# Autodesk Inventor assembly: copy2
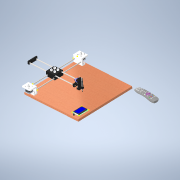
[picture p0: Inventor's stored thumbnail of the model, 180x180]
Saved by Autodesk Inventor 2021 (Build 250183000, 183)
## iProperties
Created: 2021-07-13
Part Number: copy2
Document SubType Name: Assembly
Designer: Michael Swaminathan
Author: Michael Swaminathan
## Documents named in this file (20)
- F:\Pattern Drawing Bot\Xy plotter Drawing Machine\XY Plotter Drawing Machine.iam
- F:\Pattern Drawing Bot\Xy plotter Drawing Machine\base.ipt
- F:\Pattern Drawing Bot\Xy plotter Drawing Machine\Display Controller LCD.ipt
- F:\Pattern Drawing Bot\Xy plotter Drawing Machine\Buzzer.ipt
- F:\Pattern Drawing Bot\Xy plotter Drawing Machine\Motor With Support Assembly.iam
- F:\Pattern Drawing Bot\Xy plotter Drawing Machine\Guidance Rods 2.ipt
- F:\Pattern Drawing Bot\Xy plotter Drawing Machine\Central Portion Assembly.iam
- F:\Pattern Drawing Bot\Xy plotter Drawing Machine\Y-Axis.ipt
- F:\Pattern Drawing Bot\Xy plotter Drawing Machine\Y-axis on Holder.ipt
- F:\Pattern Drawing Bot\Xy plotter Drawing Machine\Screw(2).ipt
- F:\Pattern Drawing Bot\Xy plotter Drawing Machine\Guidance Rods.ipt
- F:\Pattern Drawing Bot\Xy plotter Drawing Machine\Pen Holder.ipt
- F:\Pattern Drawing Bot\Xy plotter Drawing Machine\Holding Stand.ipt
- F:\Pattern Drawing Bot\Xy plotter Drawing Machine\BIC Round Stic Pen Assembly.iam
- F:\Pattern Drawing Bot\Xy plotter Drawing Machine\Servo Motor Support.ipt
- F:\Pattern Drawing Bot\Xy plotter Drawing Machine\Servo motor support rods.ipt
- F:\Pattern Drawing Bot\Xy plotter Drawing Machine\Micro Servo SG90.ipt
- F:\Pattern Drawing Bot\Xy plotter Drawing Machine\Rollers(2).ipt
- F:\Pattern Drawing Bot\Xy plotter Drawing Machine\roller support on y axis.ipt
- F:\Pattern Drawing Bot\Xy plotter Drawing Machine\remote controller.ipt
## Components (28 placed, 19 different names)
1. base:1 — Rigid:1, Rotational:1, Rotational:2, Rotational:3
2. Display Controller LCD:1 — Rigid:1, Rotational:4, Rotational:6, Rotational:7, Rotational:11
3. Buzzer:1 — Rotational:1
4. Motor With Support Assembly:1 [sub-assembly] — Rotational:2, Rigid:2, Rigid:3
5. Motor With Support Assembly:2 [sub-assembly] — Rotational:3, Mate:3, Mate:4
6. Guidance Rods 2:1 — Rigid:3, Mate:1, Mate:4
7. Guidance Rods 2:2 — Rigid:2, Insert:1, Mate:3
8. Central Portion Assembly:1 [sub-assembly] — Insert:1, Mate:1, Insert:2, Mate:5
9. Guidance Rods 2:3 — Mate:5, Insert:6, Mate:8
10. Guidance Rods 2:4 — Insert:2, Insert:5, Insert:12
11. Y-Axis:1 — Insert:12, Mate:8
12. Y-axis on Holder:1 — Insert:5, Insert:6, Rigid:4, Rigid:5, Rigid:12, Insert:8, Mate:7, Insert:10
13. Screw(2):1 — Rotational:11
14. Screw(2):2 — Rotational:4
15. Screw(2):3 — Rotational:6
16. Screw(2):4 — Rotational:7
17. Guidance Rods:1 — Rigid:4, Insert:7
18. Guidance Rods:2 — Rigid:5, Mate:6
19. Pen Holder:1 — Rigid:13, Insert:9
20. Holding Stand:1 — Mate:6, Insert:7, Insert:9
21. BIC Round Stic Pen Assembly:1 [sub-assembly] — Rigid:13
22. Servo Motor Support:1 — Rotational:10
23. Servo motor support rods:1 — Rigid:12, Rotational:10
24. Servo motor support rods:2 — Insert:8
25. Micro Servo SG90:1 — Mate:7
26. Rollers(2):1 — Insert:11
27. roller support on y axis:1 — Insert:10, Insert:11
28. remote controller:1
## Relationships (32: Insert 10, RevoluteJoint 8, WeldJoint 7, Mate 7)
- Rigid:1 [WeldJoint]: base:1 ↔ Display Controller LCD:1
- Rotational:1 [RevoluteJoint]: base:1 ↔ Buzzer:1
- Rotational:2 [RevoluteJoint]: base:1 ↔ Motor With Support Assembly:1
- Rotational:3 [RevoluteJoint]: base:1 ↔ Motor With Support Assembly:2
- Rigid:2 [WeldJoint] (-6 mm): Motor With Support Assembly:1 ↔ Guidance Rods 2:2
- Rigid:3 [WeldJoint] (-4 mm): Motor With Support Assembly:1 ↔ Guidance Rods 2:1
- Insert:1 (-250 mm): Guidance Rods 2:2 ↔ Central Portion Assembly:1
- Mate:1: Guidance Rods 2:1 ↔ Central Portion Assembly:1
- Insert:2 (260 mm): Central Portion Assembly:1 ↔ Guidance Rods 2:4
- Mate:3: Motor With Support Assembly:2 ↔ Guidance Rods 2:2
- Mate:4: Motor With Support Assembly:2 ↔ Guidance Rods 2:1
- Mate:5: Central Portion Assembly:1 ↔ Guidance Rods 2:3
- Rotational:4 [RevoluteJoint]: Display Controller LCD:1 ↔ Screw(2):2
- Rotational:6 [RevoluteJoint]: Display Controller LCD:1 ↔ Screw(2):3
- Rotational:7 [RevoluteJoint]: Display Controller LCD:1 ↔ Screw(2):4
- Insert:5 (-10 mm): Guidance Rods 2:4 ↔ Y-axis on Holder:1
- Insert:6 (-10 mm): Guidance Rods 2:3 ↔ Y-axis on Holder:1
- Rigid:4 [WeldJoint] (8 mm): Y-axis on Holder:1 ↔ Guidance Rods:1
- Rigid:5 [WeldJoint] (8 mm): Y-axis on Holder:1 ↔ Guidance Rods:2
- Mate:6: Guidance Rods:2 ↔ Holding Stand:1
- Rigid:13 [WeldJoint] (19 mm): Pen Holder:1 ↔ BIC Round Stic Pen Assembly:1
- Insert:7 (13.5 mm): Guidance Rods:1 ↔ Holding Stand:1
- Rigid:12 [WeldJoint]: Y-axis on Holder:1 ↔ Servo motor support rods:1
- Rotational:10 [RevoluteJoint] (7.5 mm): Servo Motor Support:1 ↔ Servo motor support rods:1
- Insert:8: Y-axis on Holder:1 ↔ Servo motor support rods:2
- Mate:7: Y-axis on Holder:1 ↔ Micro Servo SG90:1
- Insert:9 (-10 mm): Pen Holder:1 ↔ Holding Stand:1
- Insert:10 (7 mm): Y-axis on Holder:1 ↔ roller support on y axis:1
- Insert:11 (1 mm): Rollers(2):1 ↔ roller support on y axis:1
- Insert:12: Guidance Rods 2:4 ↔ Y-Axis:1
- Mate:8: Guidance Rods 2:3 ↔ Y-Axis:1
- Rotational:11 [RevoluteJoint] (-2 mm): Display Controller LCD:1 ↔ Screw(2):1
